# Autodesk Inventor assembly: Wheel Sub-Assembly
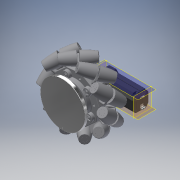
[picture p0: Inventor's stored thumbnail of the model, 180x180]
Saved by Autodesk Inventor 2019 (Build 230136000, 136)
## iProperties
Created: 2019-03-05
Part Number: Wheel Sub-Assembly
Document SubType Name: Assembly
Designer: Delta
Mass: 949.546 g
Surface Area: 3291.01 cm^2
Volume: 477.272 cm^3
Density: 1.98953 g/cm^3
Author: Delta
## Documents named in this file (7)
- C:\Robotics\2019-20_CAD\offseason\drive train\Wheel Sub-Assembly.iam
- C:\Robotics\2018-19_CAD\wheel hubcap.ipt
- C:\Robotics\COTSParts\Wheels\6inchMecanumLeft217-2799-STEP\6inchMecanumLeft217-2799.20121203.iam
- C:\Robotics\COTSParts\Rev\REV-41-1300HexMotor.ipt
- C:\Robotics\COTSParts\Rev\REV-41-1349HexAxle.ipt
- C:\Robotics\COTSParts\Vex\VersaHub 500 Hex.ipt
- C:\Robotics\COTSParts\Actobotics\545 parts\545690 assembly.ipt
## Components (6 placed, 6 different names)
1. wheel hubcap:1 — Insert:1
2. 6inchMecanumLeft217-2799.20121203:1 [sub-assembly] — Insert:1, Insert:2, Angle:1
3. REV-41-1300HexMotor:1 — Mate:2, Flush:1, Angle:2, Mate:3
4. REV-41-1349HexAxle:1 — Mate:1, Mate:2, Flush:1, Angle:2
5. VersaHub 500 Hex:1 — Insert:2, Angle:1, Insert:3
6. 545690 assembly:1 — Insert:3, Mate:1, Mate:3
## Relationships (9: Insert 3, Mate 3, Angle 2, Flush 1)
- Insert:1 (-19.431 mm): wheel hubcap:1 ↔ 6inchMecanumLeft217-2799.20121203:1
- Insert:2: 6inchMecanumLeft217-2799.20121203:1 ↔ VersaHub 500 Hex:1
- Angle:1 (0 deg): 6inchMecanumLeft217-2799.20121203:1 ↔ VersaHub 500 Hex:1
- Insert:3: VersaHub 500 Hex:1 ↔ 545690 assembly:1
- Mate:1: REV-41-1349HexAxle:1 ↔ 545690 assembly:1
- Mate:2: REV-41-1300HexMotor:1 ↔ REV-41-1349HexAxle:1
- Flush:1: REV-41-1300HexMotor:1 ↔ REV-41-1349HexAxle:1
- Angle:2 (0 deg): REV-41-1300HexMotor:1 ↔ REV-41-1349HexAxle:1
- Mate:3: REV-41-1300HexMotor:1 ↔ 545690 assembly:1
